# Autodesk Inventor assembly: Baugruppe_Poti
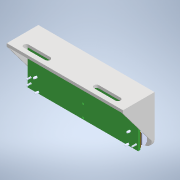
[picture p0: Inventor's stored thumbnail of the model, 180x180]
Saved by Autodesk Inventor 2022.2 (Build 262287010, 287A)
## iProperties
Created: 2024-04-03
Part Number: Baugruppe_Poti
Document SubType Name: Assembly
Designer: ppovolni
Author: ppovolni
## Documents named in this file (4)
- D:\3_Local_Projekte\ALF\alf_nmr_magnetometer\2_Project_Motiontracking_Robotarm\CAD\Potentiometer\Baugruppe_Poti.iam
- D:\3_Local_Projekte\ALF\alf_nmr_magnetometer\2_Project_Motiontracking_Robotarm\CAD\Potentiometer\Bourns_Poti.ipt
- D:\3_Local_Projekte\ALF\alf_nmr_magnetometer\2_Project_Motiontracking_Robotarm\CAD\Potentiometer\Halterung_Winkel.ipt
- D:\3_Local_Projekte\ALF\alf_nmr_magnetometer\2_Project_Motiontracking_Robotarm\CAD\Baugruppe_Braccio\4_ownParts\Poti_Sensor_PCB_.ipt
## Components (3 placed, 3 different names)
1. Bourns_Poti:1 — Fluchtend:1, Fluchtend:2, Fluchtend:3, Fluchtend:4, Fluchtend:5
2. Halterung_Winkel:1 — Fluchtend:1, Fluchtend:2
3. Poti_Sensor_PCB_:1 — Fluchtend:3, Fluchtend:4, Fluchtend:5
## Relationships (5: Flush 5)
- Fluchtend:1 [Flush]: Bourns_Poti:1 ↔ Halterung_Winkel:1
- Fluchtend:2 [Flush]: Bourns_Poti:1 ↔ Halterung_Winkel:1
- Fluchtend:3 [Flush]: Bourns_Poti:1 ↔ Poti_Sensor_PCB_:1
- Fluchtend:4 [Flush]: Bourns_Poti:1 ↔ Poti_Sensor_PCB_:1
- Fluchtend:5 [Flush]: Bourns_Poti:1 ↔ Poti_Sensor_PCB_:1
